# Autodesk Inventor assembly: Arm Assembly
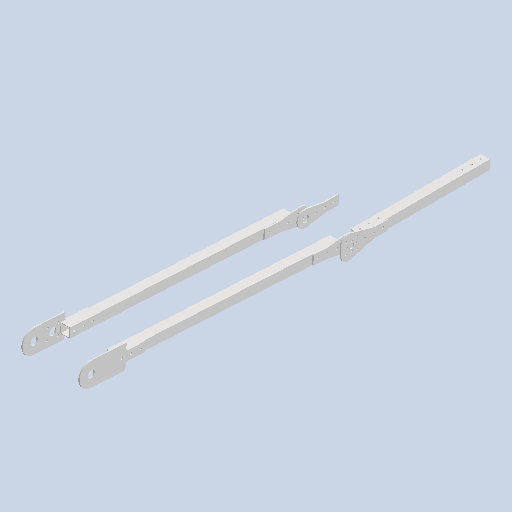
[picture p0: Inventor's stored thumbnail of the model, 512x512]
Saved by Autodesk Inventor 2025.1 (Build 291241020, 241B)
## iProperties
Created: 2024-01-10
Part Number: Arm Assembly
Document SubType Name: Assembly
Designer: david
Author: david
## Documents named in this file (8)
- C:\Users\t205b\OneDrive\Documents\Github\BehrendURCMechanical\CAD\Apparatus\ARM MAIN\Arm Assembly.iam
- C:\Users\t205b\OneDrive\Documents\Github\BehrendURCMechanical\CAD\Apparatus\ARM MAIN\Arm Plate.ipt
- C:\Users\t205b\OneDrive\Documents\Github\BehrendURCMechanical\CAD\Apparatus\ARM MAIN\Arm Plate2.ipt
- C:\Users\t205b\OneDrive\Documents\Github\BehrendURCMechanical\CAD\Apparatus\ARM MAIN\Arm Plate3.ipt
- C:\Users\t205b\OneDrive\Documents\Github\BehrendURCMechanical\CAD\Chassis V3\Wrist\wrist plate 2.ipt
- C:\Users\t205b\OneDrive\Documents\Github\BehrendURCMechanical\CAD\Chassis V3\Wrist\Wrist plate.ipt
- C:\Users\t205b\OneDrive\Documents\Github\BehrendURCMechanical\CAD\Apparatus\ARM MAIN\14in long 1in square tube.ipt
- C:\Users\t205b\OneDrive\Documents\Github\BehrendURCMechanical\CAD\Apparatus\ARM MAIN\24in long 1in square tube.ipt
## Components (10 placed, 5 different names)
1. arm plate:1 — Mate:4, Flush:9, Mate:8
2. arm plate:2 — Mate:13, Flush:13, Mate:14, Rotational:1
3. arm plate:3 — Mate:9, Flush:11, Mate:10
4. wrist plate 2:1 — Mate:17, Flush:15, Mate:18
5. Wrist plate:1 — Mate:15, Flush:14, Mate:16
6. 14in long 1in square tube:1 — Flush:1, Flush:2, Mate:5, Mate:11, Flush:12, Mate:12
7. 24in long 1in square tube:1 — Flush:3, Flush:4, Mate:4, Mate:6, Flush:9, Mate:8, Flush:10, Mate:15, Flush:14, Mate:16
8. 14in long 1in square tube:2 — Flush:1, Flush:2, Mate:5, Flush:10, Mate:9, Flush:11, Mate:10
9. 24in long 1in square tube:2 — Flush:3, Flush:4, Mate:6, Mate:13, Flush:13, Mate:14, Mate:17, Flush:15, Mate:18
10. arm plate:4 — Mate:11, Flush:12, Mate:12, Rotational:1
## Relationships (26: Mate 14, Flush 11, RevoluteJoint 1)
- Flush:1: 14in long 1in square tube:1 ↔ 14in long 1in square tube:2
- Flush:2: 14in long 1in square tube:1 ↔ 14in long 1in square tube:2
- Flush:3: 24in long 1in square tube:1 ↔ 24in long 1in square tube:2
- Flush:4: 24in long 1in square tube:1 ↔ 24in long 1in square tube:2
- Mate:4: arm plate:1 ↔ 24in long 1in square tube:1
- Mate:5 (101.6 mm): 14in long 1in square tube:1 ↔ 14in long 1in square tube:2
- Mate:6 (101.6 mm): 24in long 1in square tube:1 ↔ 24in long 1in square tube:2
- Flush:9: arm plate:1 ↔ 24in long 1in square tube:1
- Mate:8 (19.05 mm): arm plate:1 ↔ 24in long 1in square tube:1
- Flush:10 (-12.7 mm): 24in long 1in square tube:1 ↔ 14in long 1in square tube:2
- Mate:9: arm plate:3 ↔ 14in long 1in square tube:2
- Flush:11: arm plate:3 ↔ 14in long 1in square tube:2
- Mate:10 (25.4 mm): arm plate:3 ↔ 14in long 1in square tube:2
- Mate:11: 14in long 1in square tube:1 ↔ arm plate:4
- Flush:12: 14in long 1in square tube:1 ↔ arm plate:4
- Mate:12 (25.4 mm): 14in long 1in square tube:1 ↔ arm plate:4
- Mate:13: arm plate:2 ↔ 24in long 1in square tube:2
- Flush:13: arm plate:2 ↔ 24in long 1in square tube:2
- Mate:14 (19.05 mm): arm plate:2 ↔ 24in long 1in square tube:2
- Rotational:1 [RevoluteJoint] (-12.7 mm): arm plate:2 ↔ arm plate:4
- Mate:15: Wrist plate:1 ↔ 24in long 1in square tube:1
- Flush:14: Wrist plate:1 ↔ 24in long 1in square tube:1
- Mate:16 (-12.7 mm): Wrist plate:1 ↔ 24in long 1in square tube:1
- Mate:17: wrist plate 2:1 ↔ 24in long 1in square tube:2
- Flush:15: wrist plate 2:1 ↔ 24in long 1in square tube:2
- Mate:18 (-12.7 mm): wrist plate 2:1 ↔ 24in long 1in square tube:2
